# Autodesk Inventor assembly: mesoSPIM_PI_L-509_Assembly_Draft_V1
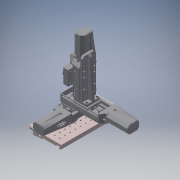
[picture p0: Inventor's stored thumbnail of the model, 180x180]
Saved by Autodesk Inventor 2016 (Build 200138000, 138)
## iProperties
Created: 2018-09-28
Part Number: mesoSPIM_PI_L-509_Assembly_Draft_V1
Document SubType Name: Assembly
Designer: voigt
Author: voigt
## Documents named in this file (7)
- D:\Microscope_Design\CAD_Files\mesoSPIM_design\mesoSPIM\sample_stages\mesoSPIM_PI_L-509_Assembly_Draft_V1.iam
- D:\Microscope_Design\CAD_Files\mesoSPIM_design\library\Qioptiq\X95_carriers\X95_300mm_carrier\X95_300mm_Carrier.iam
- D:\Microscope_Design\CAD_Files\mesoSPIM_design\library\Physik_Instrumente\L-509.20DG10.ipt
- D:\Microscope_Design\CAD_Files\mesoSPIM_design\library\Physik_Instrumente\L-509.40DG10.ipt
- D:\Microscope_Design\CAD_Files\mesoSPIM_design\library\Physik_Instrumente\KUM_L-500.AV3.ipt
- D:\Microscope_Design\CAD_Files\mesoSPIM_design\library\Physik_Instrumente\M-060.DG_KUNDENMODELL.ipt
- D:\Microscope_Design\CAD_Files\mesoSPIM_design\mesoSPIM\sample_stages\M-060-Adapter.ipt
## Components (7 placed, 6 different names)
1. X95_300mm_Carrier:1 [sub-assembly] — Mate:1, Flush:1, Flush:2
2. L-509.20DG10:1 — Mate:1, Flush:1, Flush:2, Mate:2, Mate:3, Mate:4
3. L-509.40DG10:1 — Mate:2, Mate:3, Mate:4, Mate:5, Mate:6, Mate:7
4. KUM_L-500.AV3:1 — Mate:5, Mate:6, Mate:7, Mate:8, Mate:9, Mate:10
5. L-509.20DG10:2 — Mate:8, Mate:9, Mate:10
6. M-060.DG_KUNDENMODELL:1 — Mate:11, Mate:12, Mate:13
7. M-060-Adapter:1 — Mate:11, Mate:12, Mate:13
## Relationships (15: Mate 13, Flush 2)
- Mate:1: X95_300mm_Carrier:1 ↔ L-509.20DG10:1
- Flush:1: X95_300mm_Carrier:1 ↔ L-509.20DG10:1
- Flush:2 (50 mm): X95_300mm_Carrier:1 ↔ L-509.20DG10:1
- Mate:2: L-509.20DG10:1 ↔ L-509.40DG10:1
- Mate:3: L-509.20DG10:1 ↔ L-509.40DG10:1
- Mate:4: L-509.20DG10:1 ↔ L-509.40DG10:1
- Mate:5: L-509.40DG10:1 ↔ KUM_L-500.AV3:1
- Mate:6: L-509.40DG10:1 ↔ KUM_L-500.AV3:1
- Mate:7: L-509.40DG10:1 ↔ KUM_L-500.AV3:1
- Mate:8: KUM_L-500.AV3:1 ↔ L-509.20DG10:2
- Mate:9: KUM_L-500.AV3:1 ↔ L-509.20DG10:2
- Mate:10: KUM_L-500.AV3:1 ↔ L-509.20DG10:2
- Mate:11: M-060.DG_KUNDENMODELL:1 ↔ M-060-Adapter:1
- Mate:12: M-060.DG_KUNDENMODELL:1 ↔ M-060-Adapter:1
- Mate:13: M-060.DG_KUNDENMODELL:1 ↔ M-060-Adapter:1
